# Autodesk Inventor assembly: HopperAssembly42inch_v5
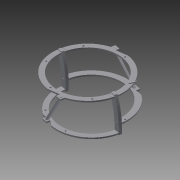
[picture p0: Inventor's stored thumbnail of the model, 180x180]
Saved by Autodesk Inventor 2013 (Build 170138000, 138)
## iProperties
Created: 2013-01-17
Part Number: HopperAssembly42inch_v5
Document SubType Name: Assembly
Designer: twsass
Mass: 496.588 g
Surface Area: 1661.96 cm^2
Volume: 413.823 cm^3
Density: 1.2 g/cm^3
Author: twsass
## Documents named in this file (8)
- C:\Users\Moses\Documents\GitHub\frc2013CAD\Launcher\Hopper\HopperAssembly42inch_v5.iam
- C:\Users\Moses\Documents\GitHub\frc2013CAD\Launcher\Hopper\TopHoopSection_v4.ipt
- C:\Users\Moses\Documents\GitHub\frc2013CAD\Launcher\Hopper\HopperFrontSupport_v2.ipt
- C:\Users\Moses\Documents\GitHub\frc2013CAD\Launcher\Hopper\BottomHoop_v1.ipt
- C:\Users\Moses\Documents\GitHub\frc2013CAD\Launcher\Hopper\MiddleHoop.ipt
- C:\Users\Moses\Documents\GitHub\frc2013CAD\Launcher\Hopper\1Piecelongsupport_v1.ipt
- C:\Users\Moses\Documents\GitHub\frc2013CAD\Launcher\Hopper\1Pieceshortsupport_v1.ipt
- C:\Users\Moses\Documents\GitHub\frc2013CAD\Launcher\Hopper\Funneling_v1.ipt
## Components (10 placed, 7 different names)
1. TopHoopSection_v4:1 — Mate:113, Mate:114, Mate:115, Flush:1, Mate:122, Mate:123, Mate:137, Mate:138, Mate:139
2. HopperFrontSupport_v2:2 — Mate:116, Mate:117, Mate:118, Mate:122, Mate:128, Mate:129, Mate:130
3. TopHoopSection_v4:2 — Mate:116, Mate:117, Mate:118, Flush:1, Mate:123, Mate:124, Mate:125, Mate:126, Mate:134, Mate:135, Mate:136
4. MiddleHoop:1 — Mate:119, Mate:120, Mate:121
5. HopperFrontSupport_v2:3 — Mate:113, Mate:114, Mate:115, Mate:119, Mate:120, Mate:121, Mate:127
6. 1Pieceshortsupport_v1:1 — Mate:124, Mate:125, Mate:126
7. BottomHoop_v1:1 — Mate:127, Mate:128, Mate:129, Mate:130, Mate:131, Mate:132, Mate:133
8. 1Piecelongsupport_v1:1 — Mate:131, Mate:132, Mate:133
9. Funneling_v1:1 — Mate:134, Mate:135, Mate:136
10. Funneling_v1:2 — Mate:137, Mate:138, Mate:139
## Relationships (28: Mate 27, Flush 1)
- Mate:113: TopHoopSection_v4:1 ↔ HopperFrontSupport_v2:3
- Mate:114: TopHoopSection_v4:1 ↔ HopperFrontSupport_v2:3
- Mate:115: TopHoopSection_v4:1 ↔ HopperFrontSupport_v2:3
- Mate:116: HopperFrontSupport_v2:2 ↔ TopHoopSection_v4:2
- Mate:117: HopperFrontSupport_v2:2 ↔ TopHoopSection_v4:2
- Mate:118: HopperFrontSupport_v2:2 ↔ TopHoopSection_v4:2
- Mate:119: MiddleHoop:1 ↔ HopperFrontSupport_v2:3
- Mate:120: MiddleHoop:1 ↔ HopperFrontSupport_v2:3
- Mate:121: MiddleHoop:1 ↔ HopperFrontSupport_v2:3
- Flush:1: TopHoopSection_v4:1 ↔ TopHoopSection_v4:2
- Mate:122: TopHoopSection_v4:1 ↔ HopperFrontSupport_v2:2
- Mate:123: TopHoopSection_v4:1 ↔ TopHoopSection_v4:2
- Mate:124: TopHoopSection_v4:2 ↔ 1Pieceshortsupport_v1:1
- Mate:125: TopHoopSection_v4:2 ↔ 1Pieceshortsupport_v1:1
- Mate:126: TopHoopSection_v4:2 ↔ 1Pieceshortsupport_v1:1
- Mate:127: HopperFrontSupport_v2:3 ↔ BottomHoop_v1:1
- Mate:128: HopperFrontSupport_v2:2 ↔ BottomHoop_v1:1
- Mate:129: HopperFrontSupport_v2:2 ↔ BottomHoop_v1:1
- Mate:130: HopperFrontSupport_v2:2 ↔ BottomHoop_v1:1
- Mate:131: BottomHoop_v1:1 ↔ 1Piecelongsupport_v1:1
- Mate:132: BottomHoop_v1:1 ↔ 1Piecelongsupport_v1:1
- Mate:133: BottomHoop_v1:1 ↔ 1Piecelongsupport_v1:1
- Mate:134: TopHoopSection_v4:2 ↔ Funneling_v1:1
- Mate:135: TopHoopSection_v4:2 ↔ Funneling_v1:1
- Mate:136: TopHoopSection_v4:2 ↔ Funneling_v1:1
- Mate:137: TopHoopSection_v4:1 ↔ Funneling_v1:2
- Mate:138: TopHoopSection_v4:1 ↔ Funneling_v1:2
- Mate:139: TopHoopSection_v4:1 ↔ Funneling_v1:2
